# Autodesk Inventor assembly: Synchronous Belts Transmission1_MIR_MIR
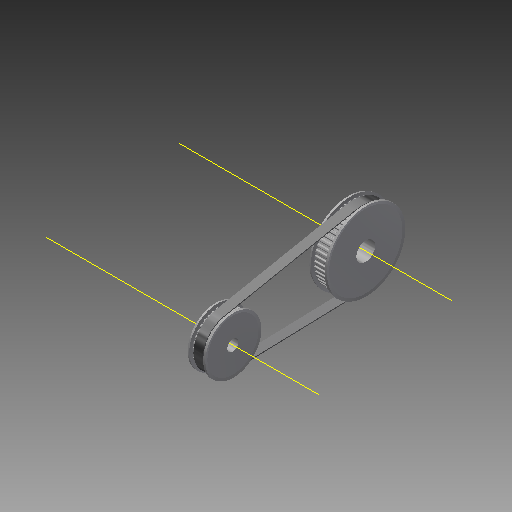
[picture p0: Inventor's stored thumbnail of the model, 512x512]
Saved by Autodesk Inventor 2019 (Build 230136000, 136)
## iProperties
Created: 2019-11-02
Part Number: Synchronous Belts Transmission1_MIR_MIR
Document SubType Name: Assembly
Designer: Mark
Author: admin
## Documents named in this file (4)
- C:\Users\Mark\Desktop\7738 Helion Engineering\7738-CAD-prep\Butterfly Drive Mk2\Butterfly Module\Butterfly Drive Module\Design Accelerator\Synchronous Belts Transmission1_MIR_MIR.iam
- C:\Users\Mark\Desktop\7738 Helion Engineering\7738-CAD-prep\Butterfly Drive Mk2\Butterfly Module\Butterfly Drive Module\Design Accelerator\Synchronous Belt1_MIR_MIR.ipt
- C:\Users\Mark\Desktop\7738 Helion Engineering\7738-CAD-prep\Butterfly Drive Mk2\Butterfly Module\Butterfly Drive Module\Design Accelerator\Synchronous Pulley11_MIR_MIR.ipt
- C:\Users\Mark\Desktop\7738 Helion Engineering\7738-CAD-prep\Butterfly Drive Mk2\Butterfly Module\Butterfly Drive Module\Design Accelerator\Synchronous Pulley21_MIR_MIR.ipt
## Components (3 placed, 3 different names)
1. Synchronous Belt1_MIR_MIR:1 — Flush:1, Mate:1, Mate:2, Flush:2, Mate:3, Mate:4
2. Synchronous Pulley11_MIR_MIR:1 — Flush:1, Mate:1, Mate:2, Rotation:1
3. Synchronous Pulley21_MIR_MIR:1 — Flush:2, Mate:3, Mate:4, Rotation:1
## Relationships (7: Mate 4, Flush 2, RelateRotation 1)
- Flush:1: Synchronous Belt1_MIR_MIR:1 ↔ Synchronous Pulley11_MIR_MIR:1
- Mate:1: Synchronous Belt1_MIR_MIR:1 ↔ Synchronous Pulley11_MIR_MIR:1
- Mate:2: Synchronous Belt1_MIR_MIR:1 ↔ Synchronous Pulley11_MIR_MIR:1
- Flush:2: Synchronous Belt1_MIR_MIR:1 ↔ Synchronous Pulley21_MIR_MIR:1
- Mate:3: Synchronous Belt1_MIR_MIR:1 ↔ Synchronous Pulley21_MIR_MIR:1
- Mate:4: Synchronous Belt1_MIR_MIR:1 ↔ Synchronous Pulley21_MIR_MIR:1
- Rotation:1 [RelateRotation] (1.4286 ul): Synchronous Pulley11_MIR_MIR:1 ↔ Synchronous Pulley21_MIR_MIR:1
